# Autodesk Inventor assembly: masbro
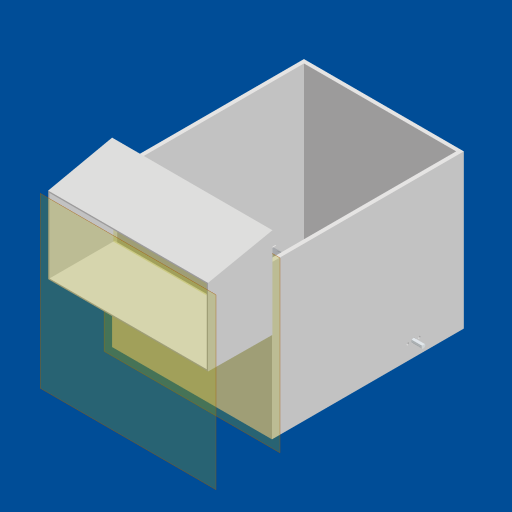
[picture p0: Inventor's stored thumbnail of the model, 512x512]
Saved by Autodesk Inventor 2023.1 (Build 271208000, 208)
## iProperties
Created: 2023-05-31
Part Number: masbro
Document SubType Name: Assembly
Designer: nara atthama
Author: nara atthama
## Documents named in this file (3)
- C:\Users\naraa\OneDrive - Universitas Airlangga\Dokumen\kuliah\MATKUL\sem6\TopSus\masbrobot\model\masbro.iam
- C:\Users\naraa\OneDrive - Universitas Airlangga\Dokumen\kuliah\MATKUL\sem6\TopSus\masbrobot\model\N20.iam
- C:\Users\naraa\OneDrive - Universitas Airlangga\Dokumen\kuliah\MATKUL\sem6\TopSus\masbrobot\model\top_case.ipt
## Components (3 placed, 2 different names)
1. N20:1 [sub-assembly] — Rotational:1, Mate:1
2. top_case:1 — Rotational:1, Mate:1, Rotational:2
3. N20:2 [sub-assembly] — Rotational:2
## Relationships (3: RevoluteJoint 2, Mate 1)
- Rotational:1 [RevoluteJoint]: N20:1 ↔ top_case:1
- Mate:1: N20:1 ↔ top_case:1
- Rotational:2 [RevoluteJoint]: top_case:1 ↔ N20:2
